# Autodesk Inventor assembly: motor unit
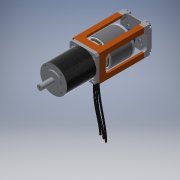
[picture p0: Inventor's stored thumbnail of the model, 180x180]
Saved by Autodesk Inventor 2018 (Build 220112000, 112)
## iProperties
Created: 2019-12-10
Part Number: motor unit
Document SubType Name: Assembly
Designer: Bunny320
Author: Bunny320
## Documents named in this file (13)
- C:\Users\Bunny320\Desktop\sechs\4-CAD\motor unit.iam
- C:\Users\Bunny320\Desktop\sechs\4-CAD\901-4250 house.ipt
- C:\Users\Bunny320\Desktop\sechs\4-CAD\911-42-reducer-long.ipt
- C:\Users\Bunny320\Desktop\sechs\4-CAD\standardParts\turnigy sk3 4250 350kv\BLDC Motor Turnigy Aerodrive SK3 350KV Outrunner.iam
- C:\Users\Bunny320\Desktop\sechs\4-CAD\902-4250 magnet hold.ipt
- C:\Users\Bunny320\Desktop\sechs\4-CAD\magnet-6x2.5.ipt
- C:\Users\Bunny320\Desktop\sechs\4-CAD\AS5047.ipt
- C:\Users\Bunny320\Desktop\sechs\4-CAD\903-4250 back.ipt
- C:\Users\Bunny320\Documents\Inventor\Content Center Files\R2018\en-US\DIN 7991(2)\DIN 7991 - M3x12.ipt
- C:\Users\Bunny320\Documents\Inventor\Content Center Files\R2018\en-US\ISO 4762(1)\DIN EN ISO 4762 - M2 x 6.ipt
- C:\Users\Bunny320\Documents\Inventor\Content Center Files\R2018\en-US\DIN EN ISO 4032\DIN EN ISO 4032 - M2.ipt
- C:\Users\Bunny320\Documents\Inventor\Content Center Files\R2018\en-US\ISO 4762(1)\DIN EN ISO 4762 - M3 x 16.ipt
- C:\Users\Bunny320\Documents\Inventor\Content Center Files\R2018\en-US\ISO 4762(1)\DIN EN ISO 4762 - M2.5 x 12.ipt
## Components (26 placed, 12 different names)
1. 901-4250 house:1 — Flush:1, Flush:2, Flush:3, Mate:1, Mate:2, Mate:3, Mate:4, Flush:4, Flush:5, Flush:6, Mate:10
2. 911-42-reducer-long:1 — Mate:3, Mate:4, Flush:4, Mate:14, Mate:15, Mate:16, Mate:17
3. BLDC Motor Turnigy Aerodrive SK3 350KV Outrunner:1 [sub-assembly] — Mate:1, Mate:2, Mate:5, Mate:6
4. 902-4250 magnet hold:1 — Mate:5, Mate:6, Mate:7, Mate:8, Insert:5, Insert:6, Insert:7
5. magnet-6x2.5:1 — Mate:7, Mate:8
6. AS5047:1 — Mate:11, Mate:12, Mate:13, Mate:19, Mate:21, Mate:23, Mate:25
7. 903-4250 back:1 — Flush:5, Flush:6, Mate:10, Mate:11, Mate:12, Mate:13, Mate:18, Mate:20, Mate:22, Mate:24, Insert:1, Insert:2, Insert:3, Insert:4, Mate:26, Mate:27, Mate:28, Mate:29, Mate:30, Mate:31, Mate:32, Mate:33
8. DIN 7991 M3x12:1 — Mate:14
9. DIN 7991 M3x12:2 — Mate:15
10. DIN 7991 M3x12:3 — Mate:16
11. DIN 7991 M3x12:4 — Mate:17
12. DIN EN ISO 4762 M2 x 6:1 — Mate:18, Mate:19
13. DIN EN ISO 4762 M2 x 6:2 — Mate:20, Mate:21
14. DIN EN ISO 4762 M2 x 6:3 — Mate:22, Mate:23
15. DIN EN ISO 4762 M2 x 6:4 — Mate:24, Mate:25
16. DIN EN ISO 4032 M2:1 — Insert:1
17. DIN EN ISO 4032 M2:2 — Insert:2
18. DIN EN ISO 4032 M2:3 — Insert:3
19. DIN EN ISO 4032 M2:4 — Insert:4
20. DIN EN ISO 4762 M3 x 16:1 — Mate:26, Mate:27
21. DIN EN ISO 4762 M3 x 16:2 — Mate:28, Mate:29
22. DIN EN ISO 4762 M3 x 16:3 — Mate:30, Mate:31
23. DIN EN ISO 4762 M3 x 16:4 — Mate:32, Mate:33
24. DIN EN ISO 4762 M2.5 x 12:1 — Insert:5
25. DIN EN ISO 4762 M2.5 x 12:2 — Insert:6
26. DIN EN ISO 4762 M2.5 x 12:3 — Insert:7
## Relationships (45: Mate 32, Insert 7, Flush 6)
- Flush:1: 901-4250 house:1
- Flush:2: 901-4250 house:1
- Flush:3: 901-4250 house:1
- Mate:1: 901-4250 house:1 ↔ BLDC Motor Turnigy Aerodrive SK3 350KV Outrunner:1
- Mate:2: 901-4250 house:1 ↔ BLDC Motor Turnigy Aerodrive SK3 350KV Outrunner:1
- Mate:3: 901-4250 house:1 ↔ 911-42-reducer-long:1
- Mate:4: 901-4250 house:1 ↔ 911-42-reducer-long:1
- Flush:4: 901-4250 house:1 ↔ 911-42-reducer-long:1
- Mate:5: BLDC Motor Turnigy Aerodrive SK3 350KV Outrunner:1 ↔ 902-4250 magnet hold:1
- Mate:6: BLDC Motor Turnigy Aerodrive SK3 350KV Outrunner:1 ↔ 902-4250 magnet hold:1
- Mate:7: 902-4250 magnet hold:1 ↔ magnet-6x2.5:1
- Mate:8: 902-4250 magnet hold:1 ↔ magnet-6x2.5:1
- Flush:5: 901-4250 house:1 ↔ 903-4250 back:1
- Flush:6: 901-4250 house:1 ↔ 903-4250 back:1
- Mate:10: 901-4250 house:1 ↔ 903-4250 back:1
- Mate:11: AS5047:1 ↔ 903-4250 back:1
- Mate:12: AS5047:1 ↔ 903-4250 back:1
- Mate:13: AS5047:1 ↔ 903-4250 back:1
- Mate:14: 911-42-reducer-long:1 ↔ DIN 7991 M3x12:1
- Mate:15: 911-42-reducer-long:1 ↔ DIN 7991 M3x12:2
- Mate:16: 911-42-reducer-long:1 ↔ DIN 7991 M3x12:3
- Mate:17: 911-42-reducer-long:1 ↔ DIN 7991 M3x12:4
- Mate:18: 903-4250 back:1 ↔ DIN EN ISO 4762 M2 x 6:1
- Mate:19: AS5047:1 ↔ DIN EN ISO 4762 M2 x 6:1
- Mate:20: 903-4250 back:1 ↔ DIN EN ISO 4762 M2 x 6:2
- Mate:21: AS5047:1 ↔ DIN EN ISO 4762 M2 x 6:2
- Mate:22: 903-4250 back:1 ↔ DIN EN ISO 4762 M2 x 6:3
- Mate:23: AS5047:1 ↔ DIN EN ISO 4762 M2 x 6:3
- Mate:24: 903-4250 back:1 ↔ DIN EN ISO 4762 M2 x 6:4
- Mate:25: AS5047:1 ↔ DIN EN ISO 4762 M2 x 6:4
- Insert:1: 903-4250 back:1 ↔ DIN EN ISO 4032 M2:1
- Insert:2: 903-4250 back:1 ↔ DIN EN ISO 4032 M2:2
- Insert:3: 903-4250 back:1 ↔ DIN EN ISO 4032 M2:3
- Insert:4: 903-4250 back:1 ↔ DIN EN ISO 4032 M2:4
- Mate:26: 903-4250 back:1 ↔ DIN EN ISO 4762 M3 x 16:1
- Mate:27: 903-4250 back:1 ↔ DIN EN ISO 4762 M3 x 16:1
- Mate:28: 903-4250 back:1 ↔ DIN EN ISO 4762 M3 x 16:2
- Mate:29: 903-4250 back:1 ↔ DIN EN ISO 4762 M3 x 16:2
- Mate:30: 903-4250 back:1 ↔ DIN EN ISO 4762 M3 x 16:3
- Mate:31: 903-4250 back:1 ↔ DIN EN ISO 4762 M3 x 16:3
- Mate:32: 903-4250 back:1 ↔ DIN EN ISO 4762 M3 x 16:4
- Mate:33: 903-4250 back:1 ↔ DIN EN ISO 4762 M3 x 16:4
- Insert:5: 902-4250 magnet hold:1 ↔ DIN EN ISO 4762 M2.5 x 12:1
- Insert:6: 902-4250 magnet hold:1 ↔ DIN EN ISO 4762 M2.5 x 12:2
- Insert:7: 902-4250 magnet hold:1 ↔ DIN EN ISO 4762 M2.5 x 12:3
